# Autodesk Inventor assembly: OnyxQuadruped
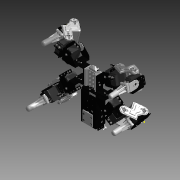
[picture p0: Inventor's stored thumbnail of the model, 180x180]
Saved by Autodesk Inventor 2015 (Build 190159000, 159)
## iProperties
Created: 2015-05-22
Part Number: OnyxQuadruped
Document SubType Name: Assembly
Designer: Quinn
Author: Quinn
## Documents named in this file (5)
- C:\Users\Quinn\Desktop\3DCNC Design\InventorModels\Assemblies\OnyxQuadruped.iam
- C:\Users\Quinn\Desktop\3DCNC Design\InventorModels\Assemblies\OnyxBody.iam
- C:\Users\Quinn\Desktop\3DCNC Design\InventorModels\Assemblies\LegAssemblyLeftRear.iam
- C:\Users\Quinn\Desktop\3DCNC Design\InventorModels\Assemblies\LegAssemblyRightFront.iam
- C:\Users\Quinn\Desktop\3DCNC Design\InventorModels\Assemblies\LegAssemblyLeftRear_MIR.iam
## Components (5 placed, 4 different names)
1. OnyxBody:1 [sub-assembly] — Rotational:1, Rotational:2, Rotational:3, Rotational:4
2. LegAssemblyLeftRear:1 [sub-assembly] — Rotational:2
3. LegAssemblyRightFront:1 [sub-assembly] — Rotational:1
4. LegAssemblyLeftRear_MIR:1 [sub-assembly] — Rotational:3
5. LegAssemblyLeftRear_MIR:2 [sub-assembly] — Rotational:4
## Relationships (4: RevoluteJoint 4)
- Rotational:1 [RevoluteJoint]: OnyxBody:1 ↔ LegAssemblyRightFront:1
- Rotational:2 [RevoluteJoint]: OnyxBody:1 ↔ LegAssemblyLeftRear:1
- Rotational:3 [RevoluteJoint]: OnyxBody:1 ↔ LegAssemblyLeftRear_MIR:1
- Rotational:4 [RevoluteJoint]: OnyxBody:1 ↔ LegAssemblyLeftRear_MIR:2
